# Autodesk Inventor assembly: main
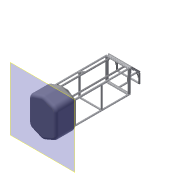
[picture p0: Inventor's stored thumbnail of the model, 180x180]
Saved by Autodesk Inventor 2014 SP1 (Build 180222100, 222)
## iProperties
Created: 2015-02-04
Part Number: main
Document SubType Name: Assembly
Designer: Simen
Author: Simen
## Documents named in this file (6)
- C:\Users\Simen\Documents\git\Eit\skjellet\main.iam
- C:\Users\Simen\Documents\git\Eit\skjellet\base.iam
- C:\Users\Simen\Documents\git\Eit\skjellet\skellett.iam
- C:\Users\Simen\Documents\git\Eit\skjellet\Head.iam
- C:\Users\Simen\Documents\git\Eit\skjellet\Head2.iam
- C:\Users\Simen\Documents\git\Eit\skjellet\KHFS5_2020_150.ipt
## Components (5 placed, 5 different names)
1. base:1 [sub-assembly] — Mate:5, Flush:16, Mate:7, Mate:8, Mate:9, Mate:10
2. skellett:1 [sub-assembly] — Mate:5, Flush:16, Flush:20, Flush:21, Mate:9, Mate:10, Flush:23, Mate:11, Flush:24, Mate:12
3. Head:1 [sub-assembly] — Flush:20, Flush:21
4. Head2:1 [sub-assembly] — Flush:23, Mate:11, Flush:24, Mate:12, Mate:13
5. KHFS5-2020-4000:1 — Mate:13
## Relationships (13: Mate 8, Flush 5)
- Mate:5: base:1 ↔ skellett:1
- Flush:16 (6 mm): base:1 ↔ skellett:1
- Mate:7: base:1
- Mate:8: base:1
- Flush:20: skellett:1 ↔ Head:1
- Flush:21: skellett:1 ↔ Head:1
- Mate:9: base:1 ↔ skellett:1
- Mate:10 (20 mm): base:1 ↔ skellett:1
- Flush:23: skellett:1 ↔ Head2:1
- Mate:11: skellett:1 ↔ Head2:1
- Flush:24: skellett:1 ↔ Head2:1
- Mate:12: skellett:1 ↔ Head2:1
- Mate:13: Head2:1 ↔ KHFS5-2020-4000:1
